# Autodesk Inventor assembly: Flex Holder V1
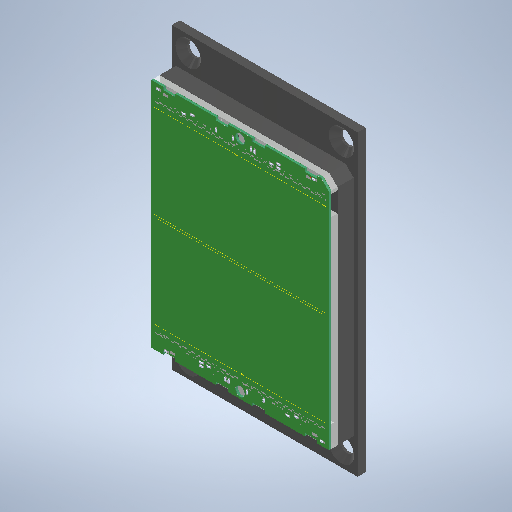
[picture p0: Inventor's stored thumbnail of the model, 512x512]
Saved by Autodesk Inventor 2025 (Build 290162000, 162)
## iProperties
Created: 2025-07-01
Part Number: Flex Holder V1
Document SubType Name: Assembly
Designer: Caleb Fangmeier
Author: Caleb Fangmeier
## Documents named in this file (4)
- C:\Users\cfang\Desktop\nebraska-silicon-lab\Hardware\ETL\Module Assembly\FLEX Holder V1\Flex Holder V1.iam
- C:\Users\cfang\Desktop\nebraska-silicon-lab\Hardware\ETL\Module Assembly\FLEX Holder V1\Flex Holder V1.ipt
- C:\Users\cfang\Desktop\nebraska-silicon-lab\Hardware\ETL\modules\Tamale v1.6\etl_etroc_module_v44\etl_etroc_module_v44.iam
- C:\Users\cfang\Desktop\nebraska-silicon-lab\Hardware\ETL\Module Assembly\FLEX Holder V1\Flex holder Base V1.ipt
## Components (3 placed, 3 different names)
1. Flex Holder V1:1 — Mate:1, Flush:1, Flush:2, Mate:2, Flush:3, Flush:4
2. etl_etroc_module_v44:1 [sub-assembly] — Mate:1, Flush:1, Flush:2
3. Flex holder Base V1:1 — Mate:2, Flush:3, Flush:4
## Relationships (6: Flush 4, Mate 2)
- Mate:1: Flex Holder V1:1 ↔ etl_etroc_module_v44:1
- Flush:1: Flex Holder V1:1 ↔ etl_etroc_module_v44:1
- Flush:2: Flex Holder V1:1 ↔ etl_etroc_module_v44:1
- Mate:2: Flex Holder V1:1 ↔ Flex holder Base V1:1
- Flush:3: Flex Holder V1:1 ↔ Flex holder Base V1:1
- Flush:4: Flex Holder V1:1 ↔ Flex holder Base V1:1
